# Autodesk Inventor assembly: MG-Straight Kicker
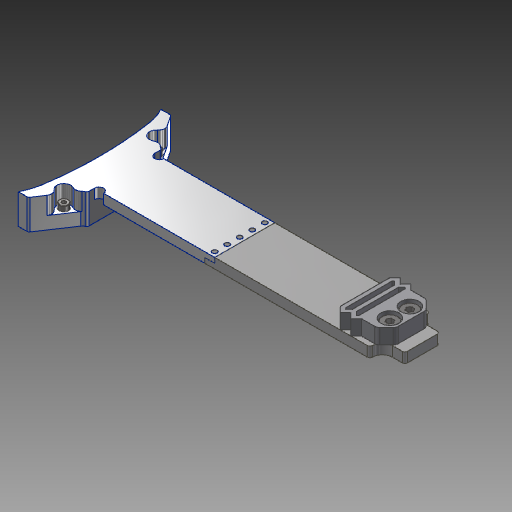
[picture p0: Inventor's stored thumbnail of the model, 512x512]
Saved by Autodesk Inventor 2019.4 (Build 234330000, 330)
## iProperties
Part Number: MG-Straight Kicker
Material: Generisch
Document SubType Name: Assembly
Designer: rYan
Mass: 83.0853 g
Surface Area: 121.113 cm^2
Volume: 18.2277 cm^3
Density: 4.5582 g/cm^3
Author: rYan
## Documents named in this file (7)
- D:\TIGERsGIT\Hardware\mechanik\2020\Inventor\Robot\Kicker\MG-Straight Kicker.iam
- D:\TIGERsGIT\Hardware\mechanik\2020\Inventor\Robot\Kicker\Kicker Eisen.ipt
- D:\TIGERsGIT\Hardware\mechanik\2020\Inventor\Purchased Parts\DIN EN ISO 2338 - 2 m6 x 4.ipt
- D:\TIGERsGIT\Hardware\mechanik\2020\Inventor\Robot\Kicker\Kicker Sichel.ipt
- D:\TIGERsGIT\Hardware\mechanik\2020\Inventor\Inhaltscenter\de-DE\ISO 4762(2)\ISO 4762 - M2 x 6ISO.ipt
- D:\TIGERsGIT\Hardware\mechanik\2020\Inventor\Robot\Kicker\Kickerdaempfer.ipt
- D:\TIGERsGIT\Hardware\mechanik\2020\Inventor\Inhaltscenter\de-DE\DIN 7984\DIN 7984 - M4 x 6.ipt
## Components (12 placed, 6 different names)
1. Kicker Sichel:1 — Fluchtend:1, Fluchtend:2, Fluchtend:3, Einfügen:1, Passend:1, Einfügen:2, Einfügen:3, Einfügen:4, Einfügen:5, Einfügen:9, Einfügen:10, Einfügen:15
2. Kicker Eisen:1 — Einfügen:1, Passend:1, Einfügen:12, Passend:2
3. DIN EN ISO 2338 - 2 m6 x 4:1 — Einfügen:2
4. DIN EN ISO 2338 - 2 m6 x 4:2 — Einfügen:3
5. DIN EN ISO 2338 - 2 m6 x 4:3 — Einfügen:4
6. DIN EN ISO 2338 - 2 m6 x 4:4 — Einfügen:5
7. ISO 4762 M2 x 6:1 — Einfügen:9
8. ISO 4762 M2 x 6:2 — Einfügen:10
9. Kickerdaempfer:1 — Einfügen:12, Passend:2, Einfügen:13, Einfügen:14
10. DIN 7984 M4 x 6:1 — Einfügen:14
11. DIN 7984 M4 x 6:2 — Einfügen:13
12. DIN EN ISO 2338 - 2 m6 x 4:5 — Einfügen:15
## Relationships (16: Insert 11, Flush 3, Mate 2)
- Fluchtend:1 [Flush]: Kicker Sichel:1
- Fluchtend:2 [Flush]: Kicker Sichel:1
- Fluchtend:3 [Flush]: Kicker Sichel:1
- Einfügen:1 [Insert]: Kicker Sichel:1 ↔ Kicker Eisen:1
- Passend:1 [Mate]: Kicker Sichel:1 ↔ Kicker Eisen:1
- Einfügen:2 [Insert]: Kicker Sichel:1 ↔ DIN EN ISO 2338 - 2 m6 x 4:1
- Einfügen:3 [Insert]: Kicker Sichel:1 ↔ DIN EN ISO 2338 - 2 m6 x 4:2
- Einfügen:4 [Insert]: Kicker Sichel:1 ↔ DIN EN ISO 2338 - 2 m6 x 4:3
- Einfügen:5 [Insert]: Kicker Sichel:1 ↔ DIN EN ISO 2338 - 2 m6 x 4:4
- Einfügen:9 [Insert] (0.5 mm): Kicker Sichel:1 ↔ ISO 4762 M2 x 6:1
- Einfügen:10 [Insert] (0.5 mm): Kicker Sichel:1 ↔ ISO 4762 M2 x 6:2
- Einfügen:12 [Insert]: Kicker Eisen:1 ↔ Kickerdaempfer:1
- Passend:2 [Mate]: Kicker Eisen:1 ↔ Kickerdaempfer:1
- Einfügen:13 [Insert]: Kickerdaempfer:1 ↔ DIN 7984 M4 x 6:2
- Einfügen:14 [Insert]: Kickerdaempfer:1 ↔ DIN 7984 M4 x 6:1
- Einfügen:15 [Insert]: Kicker Sichel:1 ↔ DIN EN ISO 2338 - 2 m6 x 4:5
